# Autodesk Inventor assembly: RT_ELE_001_ElectricalMainPlate
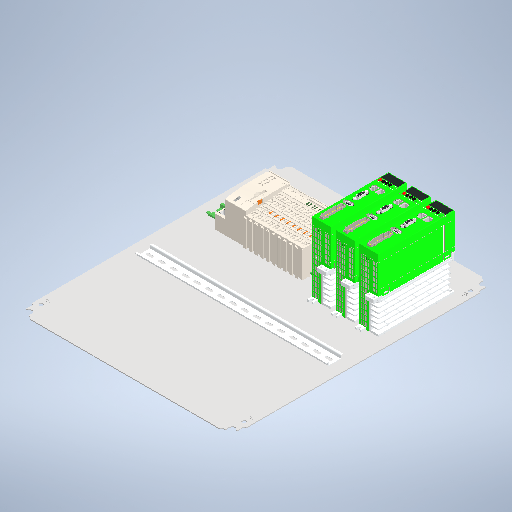
[picture p0: Inventor's stored thumbnail of the model, 512x512]
Saved by Autodesk Inventor 2025.4 (Build 294407000, 407)
## iProperties
Created: 2026-06-07
Part Number: RT_ELE_001_ElectricalMainPlate
Document SubType Name: Assembly
Designer: louis
Author: louis
## Documents named in this file (5)
- C:\Users\louis\OneDrive\Desktop\R_Trident\02_CAD\04_Subassemblies\RT_ELE_001_ElectricalMainPlate.iam
- C:\Users\louis\OneDrive\Desktop\R_Trident\02_CAD\01_Standard_Parts\04_ELE_Electrical_Automation\MCADUE0002949_3D-simplified.ipt
- C:\Users\louis\OneDrive\Desktop\R_Trident\02_CAD\01_Standard_Parts\04_ELE_Electrical_Automation\A6-400EC\A6-400EC.iam
- C:\Users\louis\OneDrive\Desktop\R_Trident\02_CAD\01_Standard_Parts\04_ELE_Electrical_Automation\LogicRail.iam
- C:\Users\louis\OneDrive\Desktop\R_Trident\02_CAD\01_Standard_Parts\04_ELE_Electrical_Automation\DIN RAIL STEEL.ipt
## Components (6 placed, 4 different names)
1. MCADUE0002949_3D-simplified:1 — Mate:1, Mate:2, Mate:3, Mate:4, Mate:5, Mate:6, Mate:7
2. A6-400EC:1 [sub-assembly] — Mate:5, Flush:2, Flush:3
3. A6-400EC:2 [sub-assembly] — Mate:4, Flush:1, Flush:2, Flush:3, Flush:4
4. A6-400EC:3 [sub-assembly] — Mate:3, Flush:1, Flush:4, Flush:10
5. LogicRail:1 [sub-assembly] — Mate:6, Flush:5
6. DIN RAIL STEEL:1 — Mate:7, Flush:5, Flush:9, Flush:10
## Relationships (14: Mate 7, Flush 7)
- Mate:1: MCADUE0002949_3D-simplified:1
- Mate:2: MCADUE0002949_3D-simplified:1
- Mate:3: MCADUE0002949_3D-simplified:1 ↔ A6-400EC:3
- Mate:4: MCADUE0002949_3D-simplified:1 ↔ A6-400EC:2
- Mate:5: MCADUE0002949_3D-simplified:1 ↔ A6-400EC:1
- Flush:1: A6-400EC:2 ↔ A6-400EC:3
- Flush:2: A6-400EC:1 ↔ A6-400EC:2
- Flush:3 (50 mm): A6-400EC:1 ↔ A6-400EC:2
- Flush:4 (50 mm): A6-400EC:2 ↔ A6-400EC:3
- Mate:6: MCADUE0002949_3D-simplified:1 ↔ LogicRail:1
- Mate:7: MCADUE0002949_3D-simplified:1 ↔ DIN RAIL STEEL:1
- Flush:5: LogicRail:1 ↔ DIN RAIL STEEL:1
- Flush:9: DIN RAIL STEEL:1
- Flush:10 (20 mm): A6-400EC:3 ↔ DIN RAIL STEEL:1
